# Autodesk Inventor assembly: 2x3
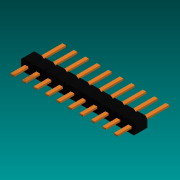
[picture p0: Inventor's stored thumbnail of the model, 180x180]
Saved by Autodesk Inventor 2015 (Build 190159000, 159)
## iProperties
Created: 2014-07-19
Part Number: 2x3
Document SubType Name: Assembly
Designer: Sawaiz Syed
Author: Sawaiz Syed
## Documents named in this file (2)
- E:\Sawaiz\3D Modeling\Projects\Radiation Dector\2.54 Breakaway\2x3.iam
- E:\Sawaiz\3D Modeling\Projects\Radiation Dector\2.54 Breakaway\1x1.iam
## Components (10 placed, 1 different names)
1. 1x1:1 [sub-assembly]
2. 1x1:2 [sub-assembly]
3. 1x1:3 [sub-assembly]
4. 1x1:4 [sub-assembly]
5. 1x1:5 [sub-assembly]
6. 1x1:6 [sub-assembly]
7. 1x1:7 [sub-assembly]
8. 1x1:8 [sub-assembly]
9. 1x1:9 [sub-assembly]
10. 1x1:10 [sub-assembly]
## Component patterns: (10 elements, first: 1x1:1)
